# Autodesk Inventor assembly: Weapon Stack
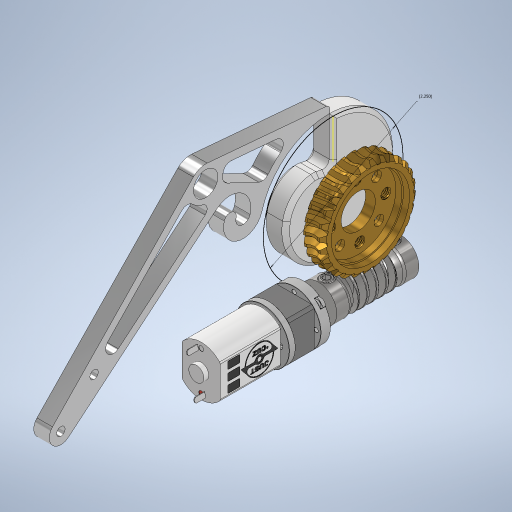
[picture p0: Inventor's stored thumbnail of the model, 512x512]
Saved by Autodesk Inventor 2023.2 (Build 272271000, 271)
## iProperties
Created: 2023-07-06
Part Number: Weapon Stack
Document SubType Name: Assembly
Designer: Nathan Cai
Author: Nathan Cai
## Documents named in this file (5)
- E:\Documents\Inventor\Flipper V0.1\Weapon Stack.iam
- E:\Documents\Inventor\Flipper V0.1\Worm Gear 28-1\Worm Gear 28-1.iam
- E:\Documents\Inventor\Flipper V0.1\Snail Cam.ipt
- E:\Documents\Inventor\Flipper V0.1\DartBox+V2+Drive+-+Just+'Cuz+Robotics\DartBox+V2+Drive+-+Just+'Cuz+Robotics.iam
- E:\Documents\Inventor\Flipper V0.1\Arm.ipt
## Components (4 placed, 4 different names)
1. Worm Gear 28-1:1 [sub-assembly] — Mate:5, Mate:6, Mate:7, Mate:8
2. Snail Cam:1 — Mate:5, Mate:6, Mate:9, Flush:1
3. DartBox+V2+Drive+-+Just+'Cuz+Robotics:1 [sub-assembly] — Mate:7, Mate:8
4. Arm:1 — Mate:9, Flush:1
## Relationships (6: Mate 5, Flush 1)
- Mate:5: Worm Gear 28-1:1 ↔ Snail Cam:1
- Mate:6 (6.35 mm): Worm Gear 28-1:1 ↔ Snail Cam:1
- Mate:7: Worm Gear 28-1:1 ↔ DartBox+V2+Drive+-+Just+'Cuz+Robotics:1
- Mate:8: Worm Gear 28-1:1 ↔ DartBox+V2+Drive+-+Just+'Cuz+Robotics:1
- Mate:9: Snail Cam:1 ↔ Arm:1
- Flush:1 (1.5875 mm): Snail Cam:1 ↔ Arm:1
